# Autodesk Inventor assembly: _PrintBoid2
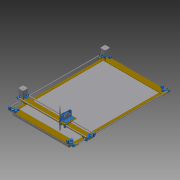
[picture p0: Inventor's stored thumbnail of the model, 180x180]
Saved by Autodesk Inventor 2013 SP2 (Build 170200200, 200)
## iProperties
Created: 2017-01-25
Part Number: _PrintBoid2
Document SubType Name: Assembly
Designer: Herman de Vries
Author: Herman de Vries
## Documents named in this file (16)
- E:\_hdv\Projects\PainterBot\_PrinterBot.iam
- E:\_hdv\Projects\PainterBot\base.ipt
- E:\_hdv\Projects\PainterBot\L Rail.ipt
- E:\_hdv\Projects\PainterBot\Z Rail assy.iam
- E:\_hdv\Projects\PainterBot\X Rail assy.iam
- E:\_hdv\Projects\PainterBot\Top Rail assy.iam
- E:\_hdv\Projects\PainterBot\Bot Rail.ipt
- E:\_hdv\Projects\PainterBot\Pully25mmx12mm.iam
- E:\_hdv\Projects\PainterBot\switch lever.ipt
- E:\_hdv\Projects\PainterBot\Pully 23mmx12mm.iam
- E:\_hdv\Projects\PainterBot\spacer top 6mm.ipt
- E:\_hdv\Projects\PainterBot\spacer 6mmx7_5mm.ipt
- E:\_hdv\Projects\PainterBot\spacer 4mmx7_5mm.ipt
- E:\_hdv\Projects\PainterBot\spacer stepperM.ipt
- E:\_hdv\Projects\PainterBot\spacer stepperM n rail.ipt
- E:\_hdv\Projects\PainterBot\y axis 8mm rod.ipt
## Components (28 placed, 15 different names)
1. base:1 — Mate:1, Flush:1, Flush:2, Mate:2, Flush:3, Flush:4, Flush:9, Flush:11
2. L Rail:1 — Mate:2, Flush:3, Flush:4
3. L Rail:2 — Mate:1, Flush:1, Flush:2, Flush:7, Flush:8, Flush:10, Mate:3, Mate:4
4. Z Rail assy:1 [sub-assembly] — Flush:12, Mate:6, Mate:7, Mate:8
5. X Rail assy:1 [sub-assembly] — Flush:11, Flush:12, Mate:6, Mate:7, Mate:8, Mate:15, Mate:16
6. Top Rail assy:1 [sub-assembly] — Flush:7, Flush:8, Mate:4, Insert:5, Insert:6, Insert:7, Insert:14, Insert:15, Insert:17, Insert:18, Mate:13
7. Bot Rail:1 — Flush:9, Flush:10, Mate:3, Mate:9, Flush:15
8. Pully 23mmx12mm:1 [sub-assembly] — Insert:12
9. Pully 23mmx12mm:2 [sub-assembly] — Insert:13
10. Pully 23mmx12mm:3 [sub-assembly] — Insert:10
11. Pully 23mmx12mm:4 [sub-assembly] — Insert:11
12. Pully25mmx12mm:1 [sub-assembly] — Insert:5, Insert:8, Insert:9
13. switch lever:1 — Insert:6, Insert:7
14. spacer top 6mm:1 — Insert:9
15. spacer 6mmx7_5mm:1 — Insert:8
16. spacer 4mmx7_5mm:1 — Insert:11
17. spacer 4mmx7_5mm:2 — Insert:10
18. spacer 4mmx7_5mm:3 — Insert:13
19. spacer 4mmx7_5mm:4 — Insert:12
20. spacer stepperM:1 — Insert:14
21. spacer stepperM:2 — Insert:15, Mate:11
22. spacer stepperM:4 — Insert:17
23. spacer stepperM n rail:1 — Insert:18, Mate:10, Mate:11, Flush:13, Insert:20
24. spacer stepperM n rail:2 — Mate:9, Mate:10, Flush:14, Flush:15
25. spacer stepperM n rail:3 — Mate:12, Mate:13, Mate:14, Flush:14
26. spacer stepperM n rail:4 — Mate:12, Mate:14, Flush:13, Insert:19
27. y axis 8mm rod:1 — Insert:19, Mate:16
28. y axis 8mm rod:2 — Insert:20, Mate:15
## Relationships (47: Insert 19, Mate 15, Flush 13)
- Mate:1: base:1 ↔ L Rail:2
- Flush:1: base:1 ↔ L Rail:2
- Flush:2: base:1 ↔ L Rail:2
- Mate:2: base:1 ↔ L Rail:1
- Flush:3: base:1 ↔ L Rail:1
- Flush:4: base:1 ↔ L Rail:1
- Flush:7 (-20 mm): L Rail:2 ↔ Top Rail assy:1
- Flush:8: L Rail:2 ↔ Top Rail assy:1
- Flush:9: base:1 ↔ Bot Rail:1
- Flush:10 (20 mm): L Rail:2 ↔ Bot Rail:1
- Mate:3: L Rail:2 ↔ Bot Rail:1
- Mate:4: L Rail:2 ↔ Top Rail assy:1
- Flush:11 (70 mm): base:1 ↔ X Rail assy:1
- Flush:12 (70 mm): Z Rail assy:1 ↔ X Rail assy:1
- [Insert] (7.5 mm): Bot Rail:1 ↔ Pully 23mmx12mm:1
- [Insert] (7.5 mm): Bot Rail:1 ↔ Pully 23mmx12mm:2
- [Insert] (7.5 mm): Bot Rail:1 ↔ Pully 23mmx12mm:4
- [Insert] (7.5 mm): Bot Rail:1 ↔ Pully 23mmx12mm:3
- Insert:5 (7.5 mm): Top Rail assy:1 ↔ Pully25mmx12mm:1
- Insert:6 (-25 mm): Top Rail assy:1 ↔ switch lever:1
- Insert:7 (-25 mm): Top Rail assy:1 ↔ switch lever:1
- Insert:8: Pully25mmx12mm:1 ↔ spacer 6mmx7_5mm:1
- Insert:9: Pully25mmx12mm:1 ↔ spacer top 6mm:1
- Insert:10: Pully 23mmx12mm:3 ↔ spacer 4mmx7_5mm:2
- Insert:11: Pully 23mmx12mm:4 ↔ spacer 4mmx7_5mm:1
- Insert:12: Pully 23mmx12mm:1 ↔ spacer 4mmx7_5mm:4
- Insert:13: Pully 23mmx12mm:2 ↔ spacer 4mmx7_5mm:3
- Insert:14: Top Rail assy:1 ↔ spacer stepperM:1
- Insert:15: Top Rail assy:1 ↔ spacer stepperM:2
- Insert:17: Top Rail assy:1 ↔ spacer stepperM:4
- Mate:6: Z Rail assy:1 ↔ X Rail assy:1
- Mate:7: Z Rail assy:1 ↔ X Rail assy:1
- Mate:8: Z Rail assy:1 ↔ X Rail assy:1
- Insert:18: Top Rail assy:1 ↔ spacer stepperM n rail:1
- Mate:9: Bot Rail:1 ↔ spacer stepperM n rail:2
- Mate:10: spacer stepperM n rail:1 ↔ spacer stepperM n rail:2
- Mate:11: spacer stepperM:2 ↔ spacer stepperM n rail:1
- Mate:12: spacer stepperM n rail:3 ↔ spacer stepperM n rail:4
- Mate:13: Top Rail assy:1 ↔ spacer stepperM n rail:3
- Mate:14: spacer stepperM n rail:3 ↔ spacer stepperM n rail:4
- Flush:13: spacer stepperM n rail:1 ↔ spacer stepperM n rail:4
- Flush:14: spacer stepperM n rail:2 ↔ spacer stepperM n rail:3
- Flush:15: Bot Rail:1 ↔ spacer stepperM n rail:2
- Insert:19: spacer stepperM n rail:4 ↔ y axis 8mm rod:1
- Insert:20: spacer stepperM n rail:1 ↔ y axis 8mm rod:2
- Mate:15: X Rail assy:1 ↔ y axis 8mm rod:2
- Mate:16: X Rail assy:1 ↔ y axis 8mm rod:1
